# Autodesk Inventor assembly: ASY Beshkino_bio_tank
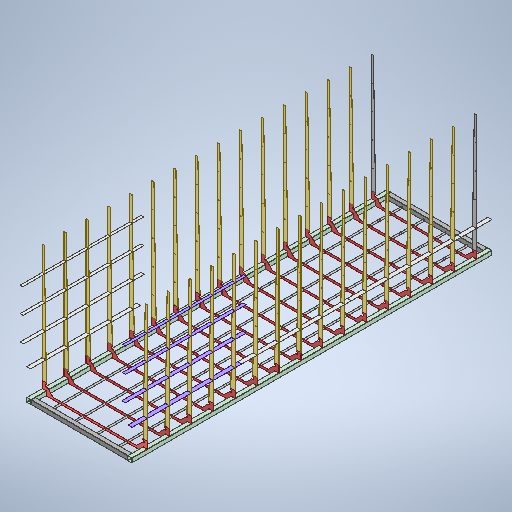
[picture p0: Inventor's stored thumbnail of the model, 512x512]
Saved by Autodesk Inventor 2025 (Build 290162010, 162A)
## iProperties
Created: 2024-07-21
Part Number: ASY Beshkino_bio_tank
Document SubType Name: Assembly
Designer: admin
Author: admin
## Documents named in this file (19)
- C:\Users\pokla\Documents\Inventor\BSH_Beshkino_bio_tank\ASY Beshkino_bio_tank.iam
- C:\Users\pokla\Documents\Inventor\BSH_Beshkino_bio_tank\BSH 000 dim Beshkino_bio_tank.ipt
- C:\Users\pokla\Documents\Inventor\BSH_Beshkino_bio_tank\BSH 010 floor 1.ipt
- C:\Users\pokla\Documents\Inventor\BSH_Beshkino_bio_tank\BSH 021 rib 1.ipt
- C:\Users\pokla\Documents\Inventor\BSH_Beshkino_bio_tank\BSH 022 rib 2.ipt
- C:\Users\pokla\Documents\Inventor\BSH_Beshkino_bio_tank\BSH 061 tube 1.ipt
- C:\Users\pokla\Documents\Inventor\BSH_Beshkino_bio_tank\BSH 031 nose 1.ipt
- C:\Users\pokla\Documents\Inventor\BSH_Beshkino_bio_tank\BSH 032 board 2.ipt
- C:\Users\pokla\Documents\Inventor\BSH_Beshkino_bio_tank\BSH 033 board 3.ipt
- C:\Users\pokla\Documents\Inventor\BSH_Beshkino_bio_tank\BSH 041 stringer 1.ipt
- C:\Users\pokla\Documents\Inventor\BSH_Beshkino_bio_tank\BSH 039 back 9.ipt
- C:\Users\pokla\Documents\Inventor\BSH_Beshkino_bio_tank\BSH 041 stringer floor.ipt
- C:\Users\pokla\Documents\Inventor\BSH_Beshkino_bio_tank\BSH 062 tube 2.ipt
- C:\Users\pokla\Documents\Inventor\BSH_Beshkino_bio_tank\BSH 042 stringer 2.ipt
- C:\Users\pokla\Documents\Inventor\BSH_Beshkino_bio_tank\BSH 043 stringer 3.ipt
- C:\Users\pokla\Documents\Inventor\BSH_Beshkino_bio_tank\BSH 044 stringer 4.ipt
- C:\Users\pokla\Documents\Inventor\BSH_Beshkino_bio_tank\BSH 020 rib 1.ipt
- C:\Users\pokla\Documents\Inventor\BSH_Beshkino_bio_tank\BSH 042 stringer floor.ipt
- C:\Users\pokla\Documents\Inventor\BSH_Beshkino_bio_tank\BSH 045 stringer 1.ipt
## Components (90 placed, 21 different names)
1. BSH 000 dim Beshkino_bio_tank.ipt:1
2. BSH 010 floor 1.ipt:1 — Mate:5, Mate:6, Rigid:4, Mate:7, Flush:4, Mate:10, Flush:5
3. BSH 022 rib 2.ipt:1 — Rigid:3, Mate:8, Rigid:27, Rigid:28, Rigid:29, Rigid:30
4. BSH 061 tube 1.ipt:1 — Mate:1, Rigid:1, Mate:3, Flush:6
5. BSH 061 tube 1.ipt:2 — Mate:2, Rigid:1, Mate:4, Flush:3, Flush:4, Rigid:14, Rigid:15, Mate:20, Mate:21
6. BSH 031 nose 1.ipt:1 — Mate:10, Flush:5, Mate:11, Rigid:11
7. BSH 010 floor 1.ipt:2 — Rigid:4, Rigid:5
8. BSH 010 floor 1.ipt:3 — Rigid:5, Rigid:6, Mate:9
9. BSH 010 floor 1.ipt:4 — Rigid:6, Rigid:7
10. BSH 010 floor 1.ipt:5 — Rigid:7, Mate:12
11. BSH 032 board 2.ipt:1 — Mate:8, Mate:9, Rigid:8
12. BSH 033 board 3.ipt:1 — Rigid:8
13. BSH 031 nose 1.ipt:2 — Rigid:11
14. BSH 041 stringer 1.ipt:1 — Rigid:27, Rigid:49
15. BSH 039 back 9.ipt:1 — Mate:12, Flush:6
16. BSH 041 stringer floor.ipt:1 — Rigid:20, Rigid:35
17. BSH 062 tube 2.ipt:1 — Rigid:14, Mate:19
18. BSH 062 tube 2.ipt:2 — Rigid:15
19. BSH 022 rib 2.ipt:2 — Rigid:16, Rigid:31, Rigid:32, Rigid:33, Rigid:34
20. BSH 021 rib 1.ipt:1 — Mate:4, Flush:3, Mate:5, Mate:6, Rigid:3, Rigid:9, Rigid:16, Rigid:20, Rigid:22, Rigid:24, Rigid:26, Mate:19
21. BSH 041 stringer floor.ipt:2 — Rigid:22, Rigid:41
22. BSH 041 stringer floor.ipt:3 — Rigid:24, Rigid:42
23. BSH 041 stringer floor.ipt:4 — Rigid:26, Rigid:43
24. BSH 042 stringer 2.ipt:1 — Rigid:28
25. BSH 043 stringer 3.ipt:1 — Rigid:29
26. BSH 044 stringer 4.ipt:1 — Rigid:30
27. BSH 041 stringer 1.ipt:2 — Rigid:31
28. BSH 042 stringer 2.ipt:2 — Rigid:32
29. BSH 043 stringer 3.ipt:2 — Rigid:33
30. BSH 044 stringer 4.ipt:2 — Rigid:34
31. BSH 041 stringer floor.ipt:5 — Rigid:35, Rigid:36
32. BSH 041 stringer floor.ipt:6 — Rigid:36
33. BSH 020 rib 1:4 — Mate:20, Mate:21, Flush:7, Rigid:37, Rigid:44, Rigid:45, Rigid:46, Rigid:47, Rigid:48
34. BSH 042 stringer floor:1 — Rigid:37
35. BSH 041 stringer floor:10 — Rigid:41
36. BSH 041 stringer floor:11
37. BSH 042 stringer floor:2 — Rigid:44
38. BSH 041 stringer floor:12 — Rigid:42
39. BSH 041 stringer floor:13
40. BSH 042 stringer floor:3 — Rigid:45
41. BSH 041 stringer floor:14 — Rigid:43
42. BSH 041 stringer floor:15
43. BSH 042 stringer floor:4 — Rigid:46
44. BSH 022 rib 2:31 — Rigid:47
45. BSH 022 rib 2:32 — Rigid:48
46. BSH 041 stringer 1:3 — Rigid:49, Rigid:50
47. BSH 041 stringer 1:4 — Rigid:50, Rigid:51
48. BSH 045 stringer 1:1 — Rigid:51
49. BSH 021 rib 1.ipt:2 — Rigid:9, Rigid:17, Rigid:18
50. BSH 022 rib 2.ipt:3 — Rigid:17
51. BSH 022 rib 2.ipt:4 — Rigid:18
52. BSH 020 rib 1:5
53. BSH 022 rib 2:5
54. BSH 022 rib 2:6
55. BSH 020 rib 1:6
56. BSH 022 rib 2:7
57. BSH 022 rib 2:8
58. BSH 020 rib 1:7
59. BSH 022 rib 2:9
60. BSH 022 rib 2:10
61. BSH 020 rib 1:8
62. BSH 022 rib 2:11
63. BSH 022 rib 2:12
64. BSH 020 rib 1:9
65. BSH 022 rib 2:13
66. BSH 022 rib 2:14
67. BSH 020 rib 1:10
68. BSH 022 rib 2:15
69. BSH 022 rib 2:16
70. BSH 020 rib 1:11
71. BSH 022 rib 2:17
72. BSH 022 rib 2:18
73. BSH 020 rib 1:12
74. BSH 022 rib 2:19
75. BSH 022 rib 2:20
76. BSH 020 rib 1:13
77. BSH 022 rib 2:21
78. BSH 022 rib 2:22
79. BSH 020 rib 1:14
80. BSH 022 rib 2:23
81. BSH 022 rib 2:24
82. BSH 020 rib 1:15
83. BSH 022 rib 2:25
84. BSH 022 rib 2:26
85. BSH 020 rib 1:16
86. BSH 022 rib 2:27
87. BSH 022 rib 2:28
88. BSH 020 rib 1:17 — Flush:7
89. BSH 022 rib 2:29
90. BSH 022 rib 2:30
## Component patterns: (14 elements, first: BSH 021 rib 1.ipt:2 + BSH 022 rib 2.ipt:3 + BSH 022 rib 2.ipt:4)
## Relationships (63: WeldJoint 43, Mate 15, Flush 5)
- Mate:1: BSH 061 tube 1.ipt:1
- Mate:2: BSH 061 tube 1.ipt:2
- Rigid:1 [WeldJoint] (-2400 mm): BSH 061 tube 1.ipt:1 ↔ BSH 061 tube 1.ipt:2
- Mate:3: BSH 061 tube 1.ipt:1
- Mate:4: BSH 061 tube 1.ipt:2 ↔ BSH 021 rib 1.ipt:1
- Flush:3: BSH 061 tube 1.ipt:2 ↔ BSH 021 rib 1.ipt:1
- Mate:5: BSH 010 floor 1.ipt:1 ↔ BSH 021 rib 1.ipt:1
- Mate:6: BSH 010 floor 1.ipt:1 ↔ BSH 021 rib 1.ipt:1
- Rigid:3 [WeldJoint]: BSH 022 rib 2.ipt:1 ↔ BSH 021 rib 1.ipt:1
- Rigid:4 [WeldJoint]: BSH 010 floor 1.ipt:1 ↔ BSH 010 floor 1.ipt:2
- Rigid:5 [WeldJoint]: BSH 010 floor 1.ipt:2 ↔ BSH 010 floor 1.ipt:3
- Rigid:6 [WeldJoint]: BSH 010 floor 1.ipt:3 ↔ BSH 010 floor 1.ipt:4
- Rigid:7 [WeldJoint]: BSH 010 floor 1.ipt:4 ↔ BSH 010 floor 1.ipt:5
- Mate:7: BSH 010 floor 1.ipt:1
- Flush:4 (100 mm): BSH 010 floor 1.ipt:1 ↔ BSH 061 tube 1.ipt:2
- Mate:8: BSH 022 rib 2.ipt:1 ↔ BSH 032 board 2.ipt:1
- Mate:9: BSH 010 floor 1.ipt:3 ↔ BSH 032 board 2.ipt:1
- Rigid:8 [WeldJoint]: BSH 032 board 2.ipt:1 ↔ BSH 033 board 3.ipt:1
- Rigid:9 [WeldJoint] (-500 mm): BSH 021 rib 1.ipt:1 ↔ BSH 021 rib 1.ipt:2
- Mate:10: BSH 010 floor 1.ipt:1 ↔ BSH 031 nose 1.ipt:1
- Flush:5 (10 mm): BSH 010 floor 1.ipt:1 ↔ BSH 031 nose 1.ipt:1
- Mate:11: BSH 031 nose 1.ipt:1
- Rigid:11 [WeldJoint]: BSH 031 nose 1.ipt:1 ↔ BSH 031 nose 1.ipt:2
- Mate:12: BSH 010 floor 1.ipt:5 ↔ BSH 039 back 9.ipt:1
- Flush:6: BSH 061 tube 1.ipt:1 ↔ BSH 039 back 9.ipt:1
- Rigid:14 [WeldJoint]: BSH 061 tube 1.ipt:2 ↔ BSH 062 tube 2.ipt:1
- Rigid:15 [WeldJoint]: BSH 061 tube 1.ipt:2 ↔ BSH 062 tube 2.ipt:2
- Rigid:16 [WeldJoint]: BSH 022 rib 2.ipt:2 ↔ BSH 021 rib 1.ipt:1
- Rigid:17 [WeldJoint]: BSH 021 rib 1.ipt:2 ↔ BSH 022 rib 2.ipt:3
- Rigid:18 [WeldJoint]: BSH 021 rib 1.ipt:2 ↔ BSH 022 rib 2.ipt:4
- Rigid:20 [WeldJoint] (2 mm): BSH 041 stringer floor.ipt:1 ↔ BSH 021 rib 1.ipt:1
- Rigid:22 [WeldJoint] (2 mm): BSH 021 rib 1.ipt:1 ↔ BSH 041 stringer floor.ipt:2
- Rigid:24 [WeldJoint]: BSH 021 rib 1.ipt:1 ↔ BSH 041 stringer floor.ipt:3
- Rigid:26 [WeldJoint] (2 mm): BSH 021 rib 1.ipt:1 ↔ BSH 041 stringer floor.ipt:4
- Rigid:27 [WeldJoint] (2 mm): BSH 022 rib 2.ipt:1 ↔ BSH 041 stringer 1.ipt:1
- Rigid:28 [WeldJoint] (2 mm): BSH 022 rib 2.ipt:1 ↔ BSH 042 stringer 2.ipt:1
- Rigid:29 [WeldJoint] (2 mm): BSH 022 rib 2.ipt:1 ↔ BSH 043 stringer 3.ipt:1
- Rigid:30 [WeldJoint] (2 mm): BSH 022 rib 2.ipt:1 ↔ BSH 044 stringer 4.ipt:1
- Rigid:31 [WeldJoint] (2 mm): BSH 022 rib 2.ipt:2 ↔ BSH 041 stringer 1.ipt:2
- Rigid:32 [WeldJoint] (2 mm): BSH 022 rib 2.ipt:2 ↔ BSH 042 stringer 2.ipt:2
- Rigid:33 [WeldJoint] (2 mm): BSH 022 rib 2.ipt:2 ↔ BSH 043 stringer 3.ipt:2
- Rigid:34 [WeldJoint] (2 mm): BSH 022 rib 2.ipt:2 ↔ BSH 044 stringer 4.ipt:2
- Mate:19 (248.5 mm): BSH 062 tube 2.ipt:1 ↔ BSH 021 rib 1.ipt:1
- Rigid:35 [WeldJoint]: BSH 041 stringer floor.ipt:1 ↔ BSH 041 stringer floor.ipt:5
- Rigid:36 [WeldJoint]: BSH 041 stringer floor.ipt:5 ↔ BSH 041 stringer floor.ipt:6
- Mate:20: BSH 061 tube 1.ipt:2 ↔ BSH 020 rib 1:4
- Mate:21: BSH 061 tube 1.ipt:2 ↔ BSH 020 rib 1:4
- Flush:7 (-500 mm): BSH 020 rib 1:4 ↔ BSH 020 rib 1:17
- Rigid:37 [WeldJoint] (2 mm): BSH 020 rib 1:4 ↔ BSH 042 stringer floor:1
- [WeldJoint]: BSH 041 stringer floor:10 ↔ BSH 041 stringer floor:11
- [WeldJoint]: BSH 041 stringer floor:12 ↔ BSH 041 stringer floor:13
- [WeldJoint]: BSH 041 stringer floor:14 ↔ BSH 041 stringer floor:15
- Rigid:41 [WeldJoint]: BSH 041 stringer floor.ipt:2 ↔ BSH 041 stringer floor:10
- Rigid:42 [WeldJoint]: BSH 041 stringer floor.ipt:3 ↔ BSH 041 stringer floor:12
- Rigid:43 [WeldJoint]: BSH 041 stringer floor.ipt:4 ↔ BSH 041 stringer floor:14
- Rigid:44 [WeldJoint] (2 mm): BSH 020 rib 1:4 ↔ BSH 042 stringer floor:2
- Rigid:45 [WeldJoint] (2 mm): BSH 020 rib 1:4 ↔ BSH 042 stringer floor:3
- Rigid:46 [WeldJoint] (2 mm): BSH 020 rib 1:4 ↔ BSH 042 stringer floor:4
- Rigid:47 [WeldJoint]: BSH 020 rib 1:4 ↔ BSH 022 rib 2:31
- Rigid:48 [WeldJoint]: BSH 020 rib 1:4 ↔ BSH 022 rib 2:32
- Rigid:49 [WeldJoint]: BSH 041 stringer 1.ipt:1 ↔ BSH 041 stringer 1:3
- Rigid:50 [WeldJoint]: BSH 041 stringer 1:3 ↔ BSH 041 stringer 1:4
- Rigid:51 [WeldJoint]: BSH 041 stringer 1:4 ↔ BSH 045 stringer 1:1
## Named parameters: d102_d89 = 0 mm, d103_d89 = 0 mm, d104_d89 = 0 mm
